# Autodesk Inventor assembly: BallJoint3mm
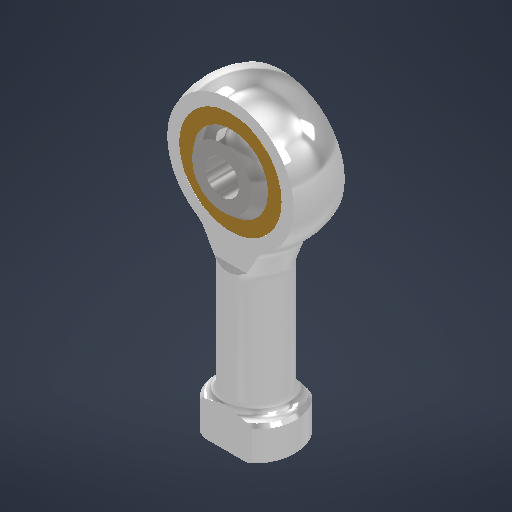
[picture p0: Inventor's stored thumbnail of the model, 512x512]
Saved by Autodesk Inventor 2025 (Build 290162000, 162)
## iProperties
Created: 2024-10-17
Part Number: BallJoint3mm
Document SubType Name: Assembly
Designer: khrip
Author: khrip
## Documents named in this file (4)
- H:\Potamon\3Dmodels\BallJoint3mm\BallJoint3mm.iam
- H:\Potamon\3Dmodels\BallJoint3mm\Parts\Ball.ipt
- H:\Potamon\3Dmodels\BallJoint3mm\Parts\Cylinder.ipt
- H:\Potamon\3Dmodels\BallJoint3mm\Parts\Body.ipt
## Components (3 placed, 3 different names)
1. Body:1 — Совмещение:1, Заподлицо:1
2. Cylinder:1 — Совмещение:1, Заподлицо:1, Совмещение:2
3. Ball:1 — Совмещение:2
## Relationships (3: Mate 2, Flush 1)
- Совмещение:1 [Mate]: Body:1 ↔ Cylinder:1
- Заподлицо:1 [Flush]: Body:1 ↔ Cylinder:1
- Совмещение:2 [Mate]: Cylinder:1 ↔ Ball:1
